# Autodesk Inventor assembly: BoBa
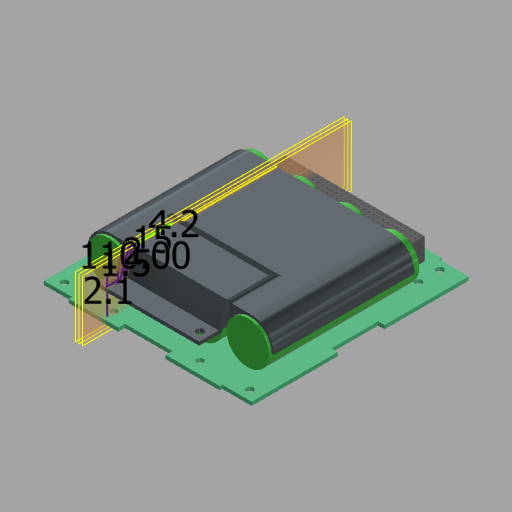
[picture p0: Inventor's stored thumbnail of the model, 512x512]
Saved by Autodesk Inventor 2022.3 (Build 263350000, 350)
## iProperties
Created: 2021-10-06
Part Number: BoBa
Document SubType Name: Assembly
Designer: Bowen O'Steen
Mass: 211.245 g
Surface Area: 553.728 cm^2
Volume: 102.991 cm^3
Density: 2.0511 g/cm^3
Author: Bowen O'Steen
## Documents named in this file (4)
- C:\Users\gwhen\OneDrive\Desktop\Vault\Designs\MEMESat\MemeSat\Engineering Data\MemeSat\Subsystems\BoBa\BoBa.iam
- C:\Users\gwhen\OneDrive\Desktop\Vault\Designs\MEMESat\MemeSat\Engineering Data\MemeSat\Subsystems\BoBa\batteriesfourpack.iam
- C:\Users\gwhen\OneDrive\Desktop\Vault\Designs\MEMESat\MemeSat\Engineering Data\MemeSat\Subsystems\blankshortpinsPC104plus.iam
- C:\Users\gwhen\OneDrive\Desktop\Vault\Designs\MEMESat\MemeSat\Engineering Data\MemeSat\Subsystems\BoBa\BobaLid.ipt
## Components (3 placed, 3 different names)
1. blankshortpinsPC104plus:1 [sub-assembly] — Mate:1, Flush:1, Mate:2, Tangent:1, Tangent:2, Mate:3, Mate:4, Tangent:3, Tangent:4
2. batteriesfourpack:1 [sub-assembly] — Tangent:1, Tangent:2, Mate:3, Mate:4, Mate:5, Mate:6
3. BobaLid:1 — Mate:5, Mate:6
## Relationships (14: Mate 6, Tangent 4, Angle 2, Flush 1, Symmetry 1)
- Mate:1: blankshortpinsPC104plus:1
- Flush:1: blankshortpinsPC104plus:1
- Mate:2: blankshortpinsPC104plus:1
- Tangent:1: blankshortpinsPC104plus:1 ↔ batteriesfourpack:1
- Tangent:2: blankshortpinsPC104plus:1 ↔ batteriesfourpack:1
- Mate:3 (5 mm): blankshortpinsPC104plus:1 ↔ batteriesfourpack:1
- Mate:4 (5 mm): blankshortpinsPC104plus:1 ↔ batteriesfourpack:1
- Mate:5: batteriesfourpack:1 ↔ BobaLid:1
- Mate:6: batteriesfourpack:1 ↔ BobaLid:1
- Angle:1 (0 deg)
- Tangent:3: blankshortpinsPC104plus:1
- Angle:2 (0 deg)
- Tangent:4: blankshortpinsPC104plus:1
- Symmetry:1
